# Autodesk Inventor assembly: ASY BSH 610 reagent dosator
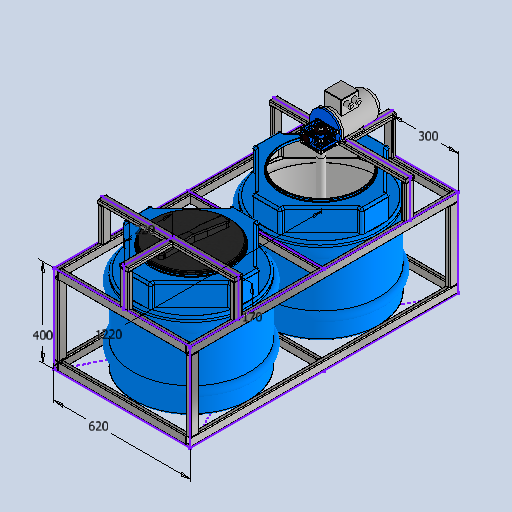
[picture p0: Inventor's stored thumbnail of the model, 512x512]
Saved by Autodesk Inventor 2025 (Build 290162010, 162A)
## iProperties
Created: 2024-09-22
Part Number: ASY BSH 610 reagent dosator
Document SubType Name: Assembly
Designer: admin
Author: admin
## Documents named in this file (7)
- C:\Users\admin\YandexDisk-badmisterfox\домашниий пк\Inventor\BSH_Beshkino_bio_tank\ASY BSH 610 reagent dosator.iam
- C:\Users\admin\YandexDisk-badmisterfox\домашниий пк\Inventor\BSH_Beshkino_bio_tank\BSH 12 reagent tank.ipt
- C:\Users\admin\YandexDisk-badmisterfox\домашниий пк\Inventor\BSH_Beshkino_bio_tank\ASY BSH tank frame.iam
- C:\Users\admin\YandexDisk-badmisterfox\домашниий пк\Inventor\BSH_Beshkino_bio_tank\1.1 крышка.ipt
- C:\Users\admin\YandexDisk-badmisterfox\домашниий пк\Inventor\BSH_Beshkino_bio_tank\3d party\reductor NMRV30\Редуктор NMRV-030.ipt
- C:\Users\admin\YandexDisk-badmisterfox\домашниий пк\Inventor\BSH_Beshkino_bio_tank\3d party\motor B4 6201-2rz  0.18kW.ipt
- C:\Users\admin\YandexDisk-badmisterfox\домашниий пк\Inventor\BSH_Beshkino_bio_tank\3d party\Mixer 22.04.24\ASY mixer 3.iam
## Components (7 placed, 6 different names)
1. ASY BSH tank frame:1 [sub-assembly] — Tangent:1, Tangent:2, Mate:5, Angle:1
2. BSH 12 reagent tank:2 — Mate:2, Mate:3, Tangent:2, Mate:6
3. BSH 12 reagent tank:1 — Mate:1, Mate:4, Tangent:1, Rotational:2
4. 1.1 крышка:1 — Rotational:2
5. NMRV-030:1 — Rigid:1, Mate:6, Rotational:3
6. motor B4 6201-2rz  0.18kW:1 — Rigid:1, Mate:5, Angle:1
7. ASY mixer 3:1 [sub-assembly] — Rotational:3
## Relationships (12: Mate 6, Tangent 2, RevoluteJoint 2, WeldJoint 1, Angle 1)
- Mate:1: BSH 12 reagent tank:1
- Mate:2: BSH 12 reagent tank:2
- Mate:3: BSH 12 reagent tank:2
- Mate:4: BSH 12 reagent tank:1
- Tangent:1: ASY BSH tank frame:1 ↔ BSH 12 reagent tank:1
- Tangent:2: ASY BSH tank frame:1 ↔ BSH 12 reagent tank:2
- Rigid:1 [WeldJoint]: NMRV-030:1 ↔ motor B4 6201-2rz  0.18kW:1
- Mate:5: ASY BSH tank frame:1 ↔ motor B4 6201-2rz  0.18kW:1
- Mate:6: BSH 12 reagent tank:2 ↔ NMRV-030:1
- Rotational:2 [RevoluteJoint]: BSH 12 reagent tank:1 ↔ 1.1 крышка:1
- Rotational:3 [RevoluteJoint]: NMRV-030:1 ↔ ASY mixer 3:1
- Angle:1 (0 deg): ASY BSH tank frame:1 ↔ motor B4 6201-2rz  0.18kW:1
